# Autodesk Inventor assembly: SmolClawAssembly
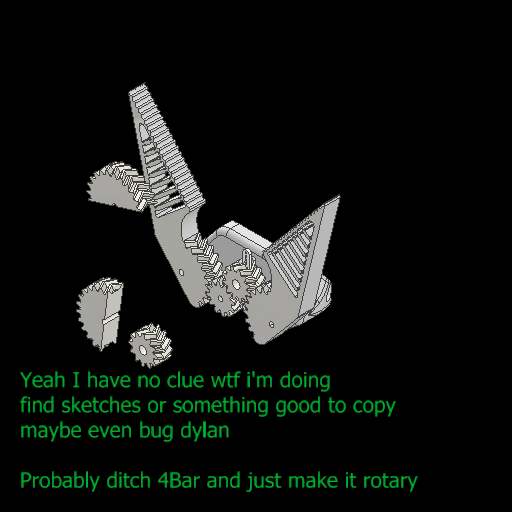
[picture p0: Inventor's stored thumbnail of the model, 512x512]
Saved by Autodesk Inventor 2023 (Build 270158000, 158)
## iProperties
Created: 2023-05-26
Part Number: SmolClawAssembly
Document SubType Name: Assembly
Designer: tandu
Author: tandu
## Documents named in this file (8)
- C:\Users\tandu\Documents\GrabCAD\Robotic Arm Project\Smol Version\V1\Claw\SmolClawAssembly.iam
- C:\Users\tandu\Documents\GrabCAD\Robotic Arm Project\Smol Version\V1\Claw\ClawServoBase.ipt
- C:\Users\tandu\Documents\GrabCAD\Robotic Arm Project\Smol Version\V1\SG90 Assembly.iam
- C:\Users\tandu\Documents\GrabCAD\Robotic Arm Project\Smol Version\V1\Claw\SmolClawAssembly\Design Accelerator\ClawGears.iam
- C:\Users\tandu\Documents\GrabCAD\Robotic Arm Project\Smol Version\V1\Claw\SmolClawAssembly\Design Accelerator\ClawGear1.ipt
- C:\Users\tandu\Documents\GrabCAD\Robotic Arm Project\Smol Version\V1\Claw\SmolClawAssembly\Design Accelerator\ClawGear2.ipt
- C:\Users\tandu\Documents\GrabCAD\Robotic Arm Project\Smol Version\V1\Claw\SmolClawAssembly\Design Accelerator\ClawGear1But3mm.ipt
- C:\Users\tandu\Documents\GrabCAD\Robotic Arm Project\Smol Version\V1\Claw\Linkage Claw2.ipt
## Components (8 placed, 7 different names)
1. ClawServoBase:1 — Insert:9, Insert:10, Insert:12, Insert:13, Insert:14
2. SG90 Assembly:1 [sub-assembly] — Insert:9, Insert:10, Insert:11
3. ClawGears:1 [sub-assembly]
4. ClawGear1:1 — Insert:11, Rotation:1, Rotation:2
5. ClawGear2:1
6. ClawGear1But3mm:1 — Insert:12, Rotation:1
7. Linkage Claw2:1 — Insert:13, Angle:1, Rotation:3
8. Linkage Claw2:2 — Insert:14, Angle:1, Rotation:2, Rotation:3
## Relationships (10: Insert 6, RelateRotation 3, Angle 1)
- Insert:9: ClawServoBase:1 ↔ SG90 Assembly:1
- Insert:10: ClawServoBase:1 ↔ SG90 Assembly:1
- Insert:11: SG90 Assembly:1 ↔ ClawGear1:1
- Insert:12 (1.1 mm): ClawServoBase:1 ↔ ClawGear1But3mm:1
- Insert:13 (1.1 mm): ClawServoBase:1 ↔ Linkage Claw2:1
- Insert:14 (1.1 mm): ClawServoBase:1 ↔ Linkage Claw2:2
- Angle:1 (180 deg): Linkage Claw2:1 ↔ Linkage Claw2:2
- Rotation:1 [RelateRotation] (1 ul): ClawGear1:1 ↔ ClawGear1But3mm:1
- Rotation:2 [RelateRotation] (0.5 ul): ClawGear1:1 ↔ Linkage Claw2:2
- Rotation:3 [RelateRotation] (1 ul): Linkage Claw2:1 ↔ Linkage Claw2:2
